# Autodesk Inventor assembly: sg90 long claw
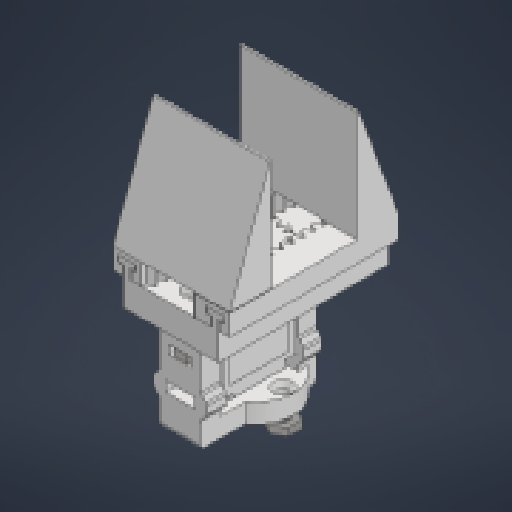
[picture p0: Inventor's stored thumbnail of the model, 512x512]
Saved by Autodesk Inventor 2026.2 (Build 302298000, 298)
## iProperties
Created: 2025-06-09
Part Number: sg90 long claw
Document SubType Name: Assembly
Designer: gavin
Author: gavin
## Documents named in this file (7)
- D:\Github\6-DOF-Robot-Arm\3D-model\robot armT 2(CAD file)\sg90 long claw.iam
- D:\Github\6-DOF-Robot-Arm\3D-model\robot armT 2(CAD file)\9G Servo Motor SG90.ipt
- D:\Github\6-DOF-Robot-Arm\3D-model\robot armT 2(CAD file)\sg90 claw v2.ipt
- D:\Github\6-DOF-Robot-Arm\3D-model\robot armT 2(CAD file)\sg90 claw v2 gear m1.ipt
- D:\Github\6-DOF-Robot-Arm\3D-model\robot armT 2(CAD file)\sg90 claw v2 holder.ipt
- D:\Github\6-DOF-Robot-Arm\3D-model\robot armT 2(CAD file)\sg90 claw finger long.ipt
- D:\Github\6-DOF-Robot-Arm\3D-model\robot armT 2(CAD file)\AS 1474 - M4(1).ipt
## Components (10 placed, 6 different names)
1. 9G Servo Motor SG90:1 — 貼合:8, 貼合:9, 貼合:10
2. sg90 claw v2:1 — 貼合:10, 齊平:3, 齊平:4
3. sg90 claw v2 gear m1:1
4. sg90 claw v2 holder:1 — 貼合:8, 貼合:9, 剛性:5, 剛性:6
5. sg90 claw finger long:1 — 齊平:3
6. sg90 claw finger long:2 — 齊平:4
7. AS 1474 - M4(1):1
8. AS 1474 - M4(1):2
9. AS 1474 - M4(1):3 — 剛性:6
10. AS 1474 - M4(1):4 — 剛性:5
## Relationships (16: Mate 10, Flush 4, WeldJoint 2)
- [Flush]: 9G Servo Motor SG90:1 ↔ sg90 claw v2:1
- [Mate]: 9G Servo Motor SG90:1 ↔ sg90 claw v2 gear m1:1
- [Mate]: 9G Servo Motor SG90:1 ↔ sg90 claw v2 gear m1:1
- [Mate]: 9G Servo Motor SG90:1 ↔ sg90 claw v2:1
- [Flush]: 9G Servo Motor SG90:1 ↔ sg90 claw v2 holder:1
- [Mate]: sg90 claw v2:1 ↔ sg90 claw finger long:1
- [Mate] (0.2 mm): sg90 claw v2:1 ↔ sg90 claw finger long:1
- [Mate]: sg90 claw v2:1 ↔ sg90 claw finger long:2
- [Mate] (0.2 mm): sg90 claw v2:1 ↔ sg90 claw finger long:2
- 貼合:8 [Mate]: 9G Servo Motor SG90:1 ↔ sg90 claw v2 holder:1
- 貼合:9 [Mate]: 9G Servo Motor SG90:1 ↔ sg90 claw v2 holder:1
- 貼合:10 [Mate]: 9G Servo Motor SG90:1 ↔ sg90 claw v2:1
- 齊平:3 [Flush]: sg90 claw v2:1 ↔ sg90 claw finger long:1
- 齊平:4 [Flush]: sg90 claw v2:1 ↔ sg90 claw finger long:2
- 剛性:5 [WeldJoint]: sg90 claw v2 holder:1 ↔ AS 1474 - M4(1):4
- 剛性:6 [WeldJoint]: sg90 claw v2 holder:1 ↔ AS 1474 - M4(1):3
